# Autodesk Inventor assembly: test_wrist
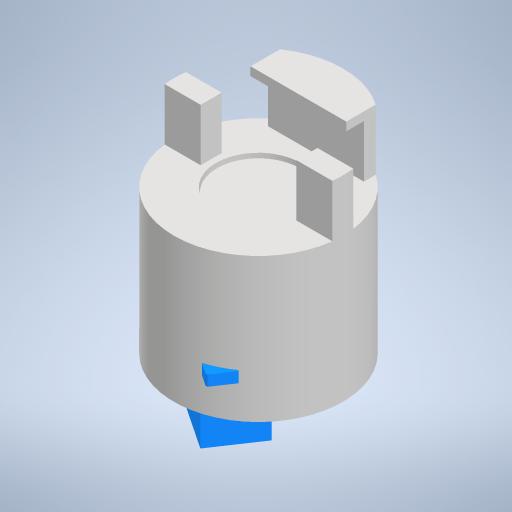
[picture p0: Inventor's stored thumbnail of the model, 512x512]
Saved by Autodesk Inventor 2024.1 (Build 281209000, 209)
## iProperties
Created: 2025-01-23
Part Number: test_wrist
Document SubType Name: Assembly
Designer: hibik
Author: hibik
## Documents named in this file (6)
- C:\Users\hibik\Documents\Robomech\RESCUE\ORCA\hard\arm\test_wrist.iam
- C:\Users\hibik\Documents\Robomech\RESCUE\ORCA\hard\arm\wrist_wrist.ipt
- C:\Users\hibik\Documents\Robomech\RESCUE\ORCA\hard\std_parts\bearing_6_10_3.ipt
- C:\Users\hibik\Documents\Robomech\RESCUE\ORCA\hard\arm\wrist_geard_hone.ipt
- C:\Users\hibik\Documents\Robomech\RESCUE\ORCA\hard\std_parts\Miusei_ms18.ipt
- C:\Users\hibik\Documents\Robomech\RESCUE\ORCA\hard\arm\wrist_hone_upper_cover.ipt
## Components (5 placed, 5 different names)
1. wrist_wrist:1 — 挿入:4
2. bearing_6_10_3:1 — 挿入:2, 挿入:5
3. wrist_geard_hone:1 — 挿入:2, 挿入:3
4. Miusei_ms18:1 — 挿入:3
5. wrist_hone_upper_cover:1 — 挿入:4, 挿入:5
## Relationships (4: Insert 4)
- 挿入:2 [Insert]: bearing_6_10_3:1 ↔ wrist_geard_hone:1
- 挿入:3 [Insert]: wrist_geard_hone:1 ↔ Miusei_ms18:1
- 挿入:4 [Insert]: wrist_wrist:1 ↔ wrist_hone_upper_cover:1
- 挿入:5 [Insert]: bearing_6_10_3:1 ↔ wrist_hone_upper_cover:1
